# Autodesk Inventor assembly: CSF-17-XXX-2UH
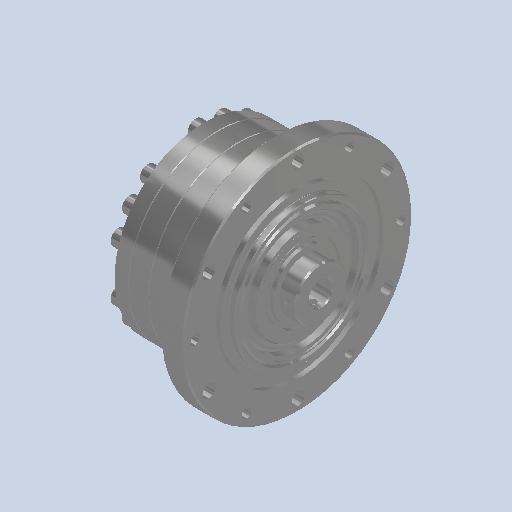
[picture p0: Inventor's stored thumbnail of the model, 512x512]
Saved by Autodesk Inventor 2025 (Build 290162000, 162)
## iProperties
Created: 2016-07-14
Part Number: CSF-17-XXX-2UH
Description: STEP AP203
Document SubType Name: Assembly
Designer: yshis
Sending System: SolidWorks 2015
Preprocessor: SwSTEP 2.0
Title: CSF-17-XXX-2UH.STEP
Revision Number: ANY
## Documents named in this file (6)
- C:\Users\yshis\Documents\ysfgit\Inventor Files\CSF-17-XXX-2UH.iam
- C:\Users\yshis\Downloads\CSF-17-XXX-2UH\CSF-17-2UH HOUSING.ipt
- C:\Users\yshis\Downloads\CSF-17-XXX-2UH\CSF-17-2UH OUTPUT.ipt
- C:\Users\yshis\Downloads\CSF-17-XXX-2UH\CSF-17-2A-R OLDHAM COUPLING.ipt
- C:\Users\yshis\Downloads\CSF-17-XXX-2UH\1715063_1715063.ipt
- C:\Users\yshis\Downloads\CSF-17-XXX-2UH\17 WG BEARING.ipt
## Components (6 placed, 6 different names)
1. CSF-17-2UH HOUSING_1
2. CSF-17-2UH OUTPUT_2
3. CSF-17-2A-R OLDHAM COUPLING_3
4. 1715063_1715063_4
5. 1715063_1715063_5
6. 17 WG BEARING_6
## Named parameters: Finish1_Area = 479.942
note: some values were not read from the file. Shown as the stored number, unit unknown: "Finish1_Area".
